# Autodesk Inventor assembly: Bolt&nut
Saved by Autodesk Inventor 2015 SP1 (Build 190203100, 203)
## iProperties
Created: 2015-01-23
Part Number: Bolt&nut
Document SubType Name: Assembly
Designer: 55221
Author: 55221
## Documents named in this file (3)
- Z:\RoboEaglesCAD\Bolt&nut.iam
- Z:\RoboEaglesCAD\wheelBase\10-24 Hex Washer Rolling x 1.25.ipt
- Z:\RoboEaglesCAD\wheelBase\10-32 Nylock Nut.ipt
## Components (2 placed, 2 different names)
1. 10-24 Hex Washer Rolling x 1.25:1
2. 10-32 Nylock Nut:1
## Relationships (1: Mate 1)
- [Mate]: 10-24 Hex Washer Rolling x 1.25:1 ↔ 10-32 Nylock Nut:1
## Named parameters: d99_d72 = 0 mm
